# Autodesk Inventor assembly: Full Small Tentacle
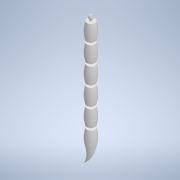
[picture p0: Inventor's stored thumbnail of the model, 180x180]
Saved by Autodesk Inventor 2021 (Build 250183000, 183)
## iProperties
Created: 2020-07-13
Part Number: Full Small Tentacle
Document SubType Name: Assembly
Designer: saipr
Author: saipr
## Documents named in this file (3)
- C:\Users\saipr\Desktop\Autodesk 2021\Builds\Parts\Samller Octopus\Full Small Tentacle.iam
- C:\Users\saipr\Desktop\Autodesk 2021\Builds\Parts\Samller Octopus\Tentalce Part.ipt
- C:\Users\saipr\Desktop\Autodesk 2021\Builds\Parts\Samller Octopus\Tentacle part end.ipt
## Components (6 placed, 2 different names)
1. Tentalce Part:1 — Mate:1, Mate:2
2. Tentalce Part:2 — Mate:2, Mate:3
3. Tentalce Part:3 — Mate:3, Mate:4
4. Tentalce Part:4 — Mate:4, Mate:5
5. Tentalce Part:5 — Mate:1
6. Tentacle part end:1 — Mate:5
## Relationships (5: Mate 5)
- Mate:1: Tentalce Part:1 ↔ Tentalce Part:5
- Mate:2: Tentalce Part:1 ↔ Tentalce Part:2
- Mate:3: Tentalce Part:2 ↔ Tentalce Part:3
- Mate:4: Tentalce Part:3 ↔ Tentalce Part:4
- Mate:5: Tentalce Part:4 ↔ Tentacle part end:1
